# Autodesk Inventor assembly: Shoulder_L
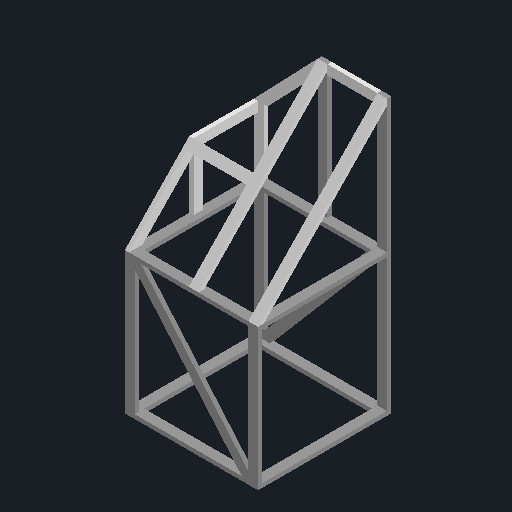
[picture p0: Inventor's stored thumbnail of the model, 512x512]
Saved by Autodesk Inventor 2026 (Build 300175000, 175)
## iProperties
Created: 2025-09-04
Part Number: Shoulder_L
Document SubType Name: Assembly
Designer: trott
Author: trott
## Documents named in this file (12)
- C:\Users\trott\Documents\UofSC-ASME-Tiger-Burn-Design-2025\CAD\Legs\Shoulder\Shoulder_R\Shoulder_R.iam
- C:\Users\trott\Documents\UofSC-ASME-Tiger-Burn-Design-2025\CAD\Legs\Front Leg\2x4x42.ipt
- C:\Users\trott\Documents\UofSC-ASME-Tiger-Burn-Design-2025\CAD\Legs\Shoulder\Shoulder_R\2x4x48.ipt
- C:\Users\trott\Documents\UofSC-ASME-Tiger-Burn-Design-2025\CAD\Legs\Shoulder\Shoulder_R\S_2x4x44.ipt
- C:\Users\trott\Documents\UofSC-ASME-Tiger-Burn-Design-2025\CAD\Legs\Shoulder\Shoulder_R\2x4x18.ipt
- C:\Users\trott\Documents\UofSC-ASME-Tiger-Burn-Design-2025\CAD\Legs\Shoulder\Shoulder_R\S_2x4x66.830.ipt
- C:\Users\trott\Documents\UofSC-ASME-Tiger-Burn-Design-2025\CAD\Legs\Shoulder\Shoulder_R\S_2x4x33.242.ipt
- C:\Users\trott\Documents\UofSC-ASME-Tiger-Burn-Design-2025\CAD\Legs\Shoulder\Shoulder_R\2x4x24.ipt
- C:\Users\trott\Documents\UofSC-ASME-Tiger-Burn-Design-2025\CAD\Legs\Shoulder\Shoulder_R\S_2x4x33.415.ipt
- C:\Users\trott\Documents\UofSC-ASME-Tiger-Burn-Design-2025\CAD\Legs\Shoulder\Shoulder_R\2x4x23.25.ipt
- C:\Users\trott\Documents\UofSC-ASME-Tiger-Burn-Design-2025\CAD\Legs\Shoulder\Shoulder_R\2x4x20.5.ipt
- C:\Users\trott\Documents\UofSC-ASME-Tiger-Burn-Design-2025\CAD\Legs\Shoulder\Shoulder_R\2x4x21.5.ipt
## Components (25 placed, 11 different names)
1. 2x4x48:3 — Mate:8, Mate:9, Mate:16, Flush:2
2. 2x4x48:4 — Mate:10, Mate:11
3. 2x4x48:5 — Mate:13, Mate:15, Mate:22
4. S_2x4x44:1 — Mate:16, Flush:2
5. S_2x4x44:2 — Mate:17, Mate:18
6. 2x4x48:9 — Mate:19, Mate:20
7. 2x4x48:10 — Mate:21, Mate:22, Mate:23, Mate:24, Mate:27
8. 2x4x18:1 — Mate:23, Mate:24, Mate:26
9. 2x4x48:11 — Mate:25, Mate:26, Mate:29, Flush:4, Mate:31, Mate:32, Flush:5
10. S_2x4x66.830:1 — Mate:29, Mate:30, Flush:4
11. S_2x4x66.830:2 — Mate:27, Mate:28, Flush:3
12. S_2x4x33.242:1 — Mate:31, Mate:32, Flush:5, Mate:35
13. 2x4x24:1 — Mate:33, Mate:34, Mate:35
14. S_2x4x33.415:1 — Mate:36, Mate:37, Mate:38, Flush:6, Mate:41, Mate:42
15. 2x4x23.25:1 — Mate:38, Flush:6, Mate:40, Mate:43
16. 2x4x20.5:1 — Mate:39, Flush:7, Mate:40
17. 2x4x21.5:1 — Mate:41, Mate:42, Mate:43
18. 2x4x42:1 — Mate:1, Flush:1, Mate:5, Mate:7
19. 2x4x48:1 — Mate:1, Flush:1, Mate:2, Mate:3, Mate:10, Mate:11, Mate:13, Mate:15
20. 2x4x48:2 — Mate:4, Mate:5, Mate:6, Mate:7, Mate:8, Mate:9, Mate:19, Mate:20
21. 2x4x42:2 — Mate:2, Mate:3, Mate:4, Mate:6, Mate:18
22. 2x4x42:3 — Mate:30
23. 2x4x48:7 — Mate:21, Mate:28, Flush:3
24. 2x4x48:8 — Mate:33, Mate:34, Mate:36, Mate:37, Mate:39, Flush:7
25. 2x4x42:4 — Mate:17, Mate:25
## Component patterns: (2 elements, first: 2x4x42:1 + 2x4x48:1 + 2x4x48:2 + 2x4x42:2)
## Relationships (48: Mate 41, Flush 7)
- Mate:1: 2x4x42:1 ↔ 2x4x48:1
- Flush:1: 2x4x42:1 ↔ 2x4x48:1
- Mate:2: 2x4x48:1 ↔ 2x4x42:2
- Mate:3: 2x4x48:1 ↔ 2x4x42:2
- Mate:4: 2x4x48:2 ↔ 2x4x42:2
- Mate:5: 2x4x42:1 ↔ 2x4x48:2
- Mate:6: 2x4x48:2 ↔ 2x4x42:2
- Mate:7: 2x4x42:1 ↔ 2x4x48:2
- Mate:8: 2x4x48:3 ↔ 2x4x48:2
- Mate:9: 2x4x48:3 ↔ 2x4x48:2
- Mate:10: 2x4x48:4 ↔ 2x4x48:1
- Mate:11: 2x4x48:4 ↔ 2x4x48:1
- Mate:13: 2x4x48:5 ↔ 2x4x48:1
- Mate:15: 2x4x48:5 ↔ 2x4x48:1
- Mate:16: 2x4x48:3 ↔ S_2x4x44:1
- Flush:2: 2x4x48:3 ↔ S_2x4x44:1
- Mate:17: S_2x4x44:2 ↔ 2x4x42:4
- Mate:18: S_2x4x44:2 ↔ 2x4x42:2
- Mate:19: 2x4x48:9 ↔ 2x4x48:2
- Mate:20: 2x4x48:9 ↔ 2x4x48:2
- Mate:21: 2x4x48:10 ↔ 2x4x48:7
- Mate:22: 2x4x48:5 ↔ 2x4x48:10
- Mate:23: 2x4x48:10 ↔ 2x4x18:1
- Mate:24: 2x4x48:10 ↔ 2x4x18:1
- Mate:25: 2x4x48:11 ↔ 2x4x42:4
- Mate:26: 2x4x18:1 ↔ 2x4x48:11
- Mate:27: 2x4x48:10 ↔ S_2x4x66.830:2
- Mate:28: S_2x4x66.830:2 ↔ 2x4x48:7
- Flush:3: S_2x4x66.830:2 ↔ 2x4x48:7
- Mate:29: 2x4x48:11 ↔ S_2x4x66.830:1
- Mate:30: S_2x4x66.830:1 ↔ 2x4x42:3
- Flush:4: 2x4x48:11 ↔ S_2x4x66.830:1
- Mate:31: 2x4x48:11 ↔ S_2x4x33.242:1
- Mate:32: 2x4x48:11 ↔ S_2x4x33.242:1
- Flush:5: 2x4x48:11 ↔ S_2x4x33.242:1
- Mate:33: 2x4x24:1 ↔ 2x4x48:8
- Mate:34: 2x4x24:1 ↔ 2x4x48:8
- Mate:35: S_2x4x33.242:1 ↔ 2x4x24:1
- Mate:36: S_2x4x33.415:1 ↔ 2x4x48:8
- Mate:37: S_2x4x33.415:1 ↔ 2x4x48:8
- Mate:38: S_2x4x33.415:1 ↔ 2x4x23.25:1
- Flush:6: S_2x4x33.415:1 ↔ 2x4x23.25:1
- Mate:39: 2x4x20.5:1 ↔ 2x4x48:8
- Flush:7: 2x4x20.5:1 ↔ 2x4x48:8
- Mate:40: 2x4x23.25:1 ↔ 2x4x20.5:1
- Mate:41: S_2x4x33.415:1 ↔ 2x4x21.5:1
- Mate:42: S_2x4x33.415:1 ↔ 2x4x21.5:1
- Mate:43: 2x4x23.25:1 ↔ 2x4x21.5:1
